# Autodesk Inventor assembly: EnsamblePie
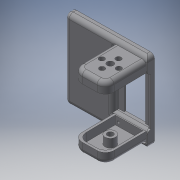
[picture p0: Inventor's stored thumbnail of the model, 180x180]
Saved by Autodesk Inventor 2019 (Build 230136000, 136)
## iProperties
Created: 2016-12-20
Part Number: EnsamblePie
Document SubType Name: Assembly
Designer: Mario
Author: Mario
## Documents named in this file (4)
- D:\Documents\Kevin\robot\EnsamblePie.iam
- D:\Documents\Kevin\robot\Pie.ipt
- D:\Documents\Kevin\robot\TapaPieEfector.ipt
- D:\Documents\Kevin\robot\TapaPieBack.ipt
## Components (3 placed, 3 different names)
1. Pie:1 — Insert:1, Angle:1
2. TapaPieEfector:1
3. TapaPieBack:1 — Insert:1, Angle:1
## Relationships (2: Insert 1, Angle 1)
- Insert:1: Pie:1 ↔ TapaPieBack:1
- Angle:1 (0 deg): Pie:1 ↔ TapaPieBack:1
